# Autodesk Inventor assembly: 5_molde_resina_mas_stock_alumnio
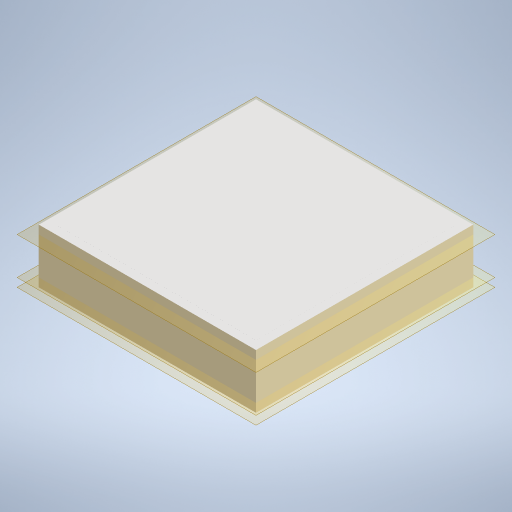
[picture p0: Inventor's stored thumbnail of the model, 512x512]
Saved by Autodesk Inventor 2023.2 (Build 272271030, 271C)
## iProperties
Created: 2023-08-30
Part Number: 5_molde_resina_mas_stock_alumnio
Document SubType Name: Assembly
Designer: Cris Pat
Author: Cris Pat
## Documents named in this file (3)
- C:\Users\Cris Pat\Desktop\U\Semestre_10\Disenio_y_manufactura\Molde_Github\5_molde_resina_mas_stock_alumnio.iam
- C:\Users\Cris Pat\Desktop\U\Semestre_10\Disenio_y_manufactura\Molde_Github\4_molde_resina.ipt
- C:\Users\Cris Pat\Desktop\U\Semestre_10\Disenio_y_manufactura\Molde_Github\STOCK_ALUMINIO.ipt
## Components (2 placed, 2 different names)
1. 4_molde_resina:1
2. STOCK_ALUMINIO:1 — Flush:1
## Relationships (1: Flush 1)
- Flush:1: STOCK_ALUMINIO:1
